# Autodesk Inventor assembly: front_bearings
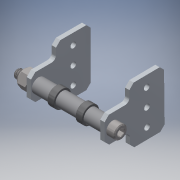
[picture p0: Inventor's stored thumbnail of the model, 180x180]
Saved by Autodesk Inventor 2018 (Build 220112000, 112)
## iProperties
Created: 2018-07-13
Part Number: front_bearings
Document SubType Name: Assembly
Designer: baoan
Author: baoan
## Documents named in this file (7)
- C:\Users\baoan\Documents\Inventor\Elevator\front_bearings.iam
- C:\Users\baoan\Documents\Inventor\Elevator\Elevator parts\McMaster-Carr 91251A553_91251A553.ipt
- C:\Users\baoan\Documents\Inventor\Elevator\217-4399-002 Rev1.ipt
- C:\Users\baoan\Documents\Inventor\Elevator\Elevator parts\217-3489-001 Rev1.ipt
- C:\Users\baoan\Documents\Inventor\Elevator\Elevator parts\McMaster-Carr 90640A129_90640A129.ipt
- C:\Users\baoan\Documents\Inventor\Elevator\0.5''_spacer.ipt
- C:\Users\baoan\Documents\Inventor\Elevator\.625''_spacer.ipt
## Components (9 placed, 6 different names)
1. McMaster-Carr 91251A553_91251A553:1 — Mate:2, Mate:3, Mate:4, Mate:5, Mate:7, Mate:9, Mate:11, Mate:13, Mate:15
2. 217-4399-002 Rev1:1 — Mate:1, Mate:3, Mate:4, Mate:8
3. 217-3489-001 Rev1:1 — Mate:9, Mate:10, Mate:12
4. 217-3489-001 Rev1:2 — Mate:13, Mate:14
5. McMaster-Carr 90640A129_90640A129:1 — Mate:5, Mate:6
6. 217-4399-002 Rev1:2 — Mate:1, Mate:2, Mate:6, Mate:16
7. 0.5''_spacer:1 — Mate:7, Mate:8, Mate:10
8. .625''_spacer:1 — Mate:11, Mate:12, Mate:14
9. 0.5''_spacer:2 — Mate:15, Mate:16
## Relationships (16: Mate 16)
- Mate:1 (50.8 mm): 217-4399-002 Rev1:1 ↔ 217-4399-002 Rev1:2
- Mate:2: McMaster-Carr 91251A553_91251A553:1 ↔ 217-4399-002 Rev1:2
- Mate:3: McMaster-Carr 91251A553_91251A553:1 ↔ 217-4399-002 Rev1:1
- Mate:4: McMaster-Carr 91251A553_91251A553:1 ↔ 217-4399-002 Rev1:1
- Mate:5: McMaster-Carr 91251A553_91251A553:1 ↔ McMaster-Carr 90640A129_90640A129:1
- Mate:6: McMaster-Carr 90640A129_90640A129:1 ↔ 217-4399-002 Rev1:2
- Mate:7: McMaster-Carr 91251A553_91251A553:1 ↔ 0.5''_spacer:1
- Mate:8: 217-4399-002 Rev1:1 ↔ 0.5''_spacer:1
- Mate:9: McMaster-Carr 91251A553_91251A553:1 ↔ 217-3489-001 Rev1:1
- Mate:10: 217-3489-001 Rev1:1 ↔ 0.5''_spacer:1
- Mate:11: McMaster-Carr 91251A553_91251A553:1 ↔ .625''_spacer:1
- Mate:12: 217-3489-001 Rev1:1 ↔ .625''_spacer:1
- Mate:13: McMaster-Carr 91251A553_91251A553:1 ↔ 217-3489-001 Rev1:2
- Mate:14: 217-3489-001 Rev1:2 ↔ .625''_spacer:1
- Mate:15: McMaster-Carr 91251A553_91251A553:1 ↔ 0.5''_spacer:2
- Mate:16: 217-4399-002 Rev1:2 ↔ 0.5''_spacer:2
